# Autodesk Inventor assembly: Expansor
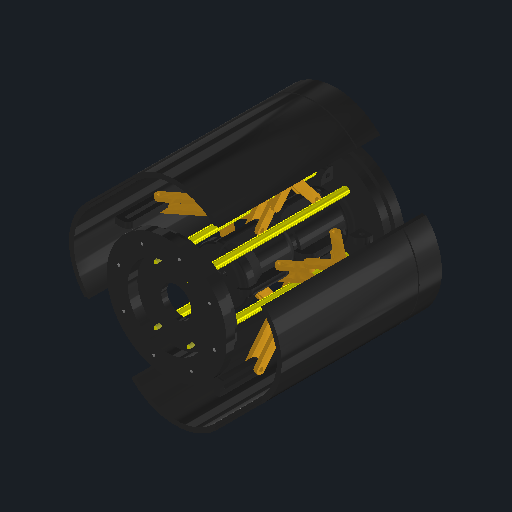
[picture p0: Inventor's stored thumbnail of the model, 512x512]
Saved by Autodesk Inventor 2025.4 (Build 294407000, 407)
## iProperties
Created: 2025-10-11
Part Number: Expansor
Document SubType Name: Assembly
Designer: santa
Author: santa
## Documents named in this file (10)
- C:\Users\danie\OneDrive\Documentos\Inventor\Arbol\V4\V4\Expansor.iam
- C:\Users\danie\OneDrive\Documentos\Inventor\Arbol\V4\V4\Expansor\Columnas.ipt
- C:\Users\danie\OneDrive\Documentos\Inventor\Arbol\V4\V4\Expansor\Corredor.ipt
- C:\Users\danie\OneDrive\Documentos\Inventor\Arbol\V4\V4\Expansor\Paletas.ipt
- C:\Users\danie\OneDrive\Documentos\Inventor\Arbol\V4\V4\Expansor\Soporte.ipt
- C:\Users\danie\OneDrive\Documentos\Inventor\Arbol\V4\V4\Expansor\Soporte2.ipt
- C:\Users\danie\OneDrive\Documentos\Inventor\Arbol\V4\V4\Expansor\Clavija.ipt
- C:\Users\danie\OneDrive\Documentos\Inventor\Arbol\V4\V4\Expansor\Corredera I.ipt
- C:\Users\danie\OneDrive\Documentos\Inventor\Arbol\V4\V4\Expansor\Corredera II.ipt
- C:\Users\danie\OneDrive\Documentos\Inventor\Arbol\V4\V4\Expansor\Columnas_MIR.ipt
## Components (23 placed, 9 different names)
1. Corredor:1 — Mate:1, Mate:2, Flush:1, Rotational:1
2. Soporte:1 — Mate:1, Mate:2, Flush:1, Mate:4, Mate:6, Mate:8, Angle:1, Tangent:2, Angle:2, Rotational:3
3. Soporte2:1 — Mate:5, Mate:6, Mate:7
4. Columnas_MIR:1
5. Columnas_MIR:2
6. Paletas:1 — Rotational:2, Tangent:3
7. Clavija:1 — Mate:12, Mate:13
8. Corredera I:1 — Rotational:1, Rotational:2, Mate:11, Mate:12
9. Corredera II:1 — Rotational:3, Mate:11, Mate:13, Tangent:3
10. Paletas:2
11. Clavija:2
12. Corredera I:2
13. Corredera II:2
14. Paletas:3
15. Clavija:3
16. Corredera I:3
17. Corredera II:3
18. Paletas:4
19. Clavija:4
20. Corredera I:4
21. Corredera II:4
22. Columnas:1 — Mate:4, Mate:5, Mate:7, Mate:8
23. Columnas:2
## Component patterns: (4 elements, first: Paletas:1 + Clavija:1 + Corredera I:1 + Corredera II:1), (2 elements, first: Columnas:1)
## Relationships (20: Mate 11, RevoluteJoint 3, Flush 2, Angle 2, Tangent 2)
- Mate:1: Corredor:1 ↔ Soporte:1
- Mate:2: Corredor:1 ↔ Soporte:1
- Flush:1: Corredor:1 ↔ Soporte:1
- Mate:4: Soporte:1 ↔ Columnas:1
- Mate:5: Soporte2:1 ↔ Columnas:1
- Mate:6: Soporte:1 ↔ Soporte2:1
- Mate:7: Soporte2:1 ↔ Columnas:1
- Mate:8: Soporte:1 ↔ Columnas:1
- Angle:1 (0 deg): Soporte:1
- Tangent:2: Soporte:1
- Mate:10
- Angle:2 (0 deg): Soporte:1
- Flush:2
- Rotational:1 [RevoluteJoint]: Corredor:1 ↔ Corredera I:1
- Rotational:2 [RevoluteJoint]: Paletas:1 ↔ Corredera I:1
- Rotational:3 [RevoluteJoint]: Soporte:1 ↔ Corredera II:1
- Mate:11: Corredera I:1 ↔ Corredera II:1
- Mate:12: Clavija:1 ↔ Corredera I:1
- Mate:13: Clavija:1 ↔ Corredera II:1
- Tangent:3: Paletas:1 ↔ Corredera II:1
